# Autodesk Inventor assembly: Thigh-40x
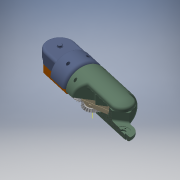
[picture p0: Inventor's stored thumbnail of the model, 180x180]
Saved by Autodesk Inventor 2018 (Build 220112000, 112)
## iProperties
Part Number: Thigh-40x
Material: Generisch
Document SubType Name: Assembly
Designer: Jochen Alt
Mass: 186.402 g
Surface Area: 1060.57 cm^2
Volume: 140.56 cm^3
Density: 1.32614 g/cm^3
Author: Jochen Alt
## Documents named in this file (12)
- D:\Projects\Manfred\design\cad\Inventor\Thigh.iam
- D:\Projects\Manfred\design\cad\Inventor\Herkulex DRS-010x\W 61707-2RS1.ipt
- D:\Projects\Manfred\design\cad\Inventor\Rillenkugellager 11x7x3 inafag smr117.ipt
- D:\Projects\Manfred\design\cad\Inventor\Thigh.ipt
- D:\Projects\Manfred\design\cad\Inventor\Herkulex DRS-040x.ipt
- D:\Projects\Manfred\design\cad\Inventor\Knee.ipt
- D:\Projects\Manfred\design\cad\Inventor\Herkulex DRS-010x\HerkuleX DRS-0101.iam
- D:\Projects\Manfred\design\cad\Inventor\Thigh Bushing.ipt
- D:\Projects\Manfred\design\cad\Inventor\ThighKneeGear.iam
- C:\Users\JochenAlt\Documents\Inventor\Content Center Files\R2018\de-DE\ISO 4762(1)\DIN EN ISO 4762 - M2 x 8.ipt
- C:\Users\JochenAlt\Documents\Inventor\Content Center Files\R2018\de-DE\ISO 4762(1)\DIN EN ISO 4762 - M2 x 6.ipt
- C:\Users\JochenAlt\Documents\Inventor\Content Center Files\R2018\de-DE\ISO 4762(1)\DIN EN ISO 4762 - M2,5 x 5.ipt
## Components (21 placed, 11 different names)
1. W 61707-2RS1:1 — Passend:44, Passend:54, Passend:73, Passend:74
2. Rillenkugellager 11x7x3 inafag smr117:2 — Passend:78, Passend:79
3. Thigh:1 — Passend:44, Passend:54, Winkel:2, Fluchtend:1, Passend:64, Winkel:3, Passend:75, Passend:77, Winkel:5, Passend:83, Einfügen:1, Einfügen:2, Einfügen:3, Einfügen:4
4. Herkulex DRS-040x:1 — Winkel:2, Fluchtend:1, Passend:64
5. Knee:1 — Passend:75, Winkel:4, Passend:82, Passend:84, Einfügen:5, Einfügen:6, Einfügen:7, Einfügen:8, Einfügen:9, Einfügen:10
6. HerkuleX DRS-0101:1 [sub-assembly] — Winkel:4, Passend:80, Passend:81
7. Thigh Bushing:1 — Passend:73, Passend:74, Passend:76, Passend:84
8. ThighKneeGear:1 [sub-assembly] — Passend:76, Passend:77, Winkel:5, Passend:78, Passend:79, Passend:80, Passend:81, Passend:82, Passend:83, Einfügen:11, Einfügen:12, Einfügen:13
9. DIN EN ISO 4762 M2,5 x 5:2 — Einfügen:1
10. DIN EN ISO 4762 M2,5 x 5:3 — Einfügen:2
11. DIN EN ISO 4762 M2,5 x 5:1 — Einfügen:3
12. DIN EN ISO 4762 M2,5 x 5:4 — Einfügen:4
13. DIN EN ISO 4762 M2 x 6:1 — Einfügen:5
14. DIN EN ISO 4762 M2 x 6:2 — Einfügen:6
15. DIN EN ISO 4762 M2 x 6:3 — Einfügen:7
16. DIN EN ISO 4762 M2 x 6:5 — Einfügen:8
17. DIN EN ISO 4762 M2 x 6:4 — Einfügen:9
18. DIN EN ISO 4762 M2 x 6:6 — Einfügen:10
19. DIN EN ISO 4762 M2 x 8:1 — Einfügen:11
20. DIN EN ISO 4762 M2 x 8:2 — Einfügen:12
21. DIN EN ISO 4762 M2 x 8:3 — Einfügen:13
## Relationships (33: Mate 15, Insert 13, Angle 4, Flush 1)
- Passend:44 [Mate]: W 61707-2RS1:1 ↔ Thigh:1
- Passend:54 [Mate]: W 61707-2RS1:1 ↔ Thigh:1
- Winkel:2 [Angle] (180 deg): Thigh:1 ↔ Herkulex DRS-040x:1
- Fluchtend:1 [Flush] (0.2 mm): Thigh:1 ↔ Herkulex DRS-040x:1
- Passend:64 [Mate]: Thigh:1 ↔ Herkulex DRS-040x:1
- Winkel:3 [Angle] (0 deg): Thigh:1
- Passend:73 [Mate]: W 61707-2RS1:1 ↔ Thigh Bushing:1
- Passend:74 [Mate] (0.1 mm): W 61707-2RS1:1 ↔ Thigh Bushing:1
- Passend:75 [Mate]: Thigh:1 ↔ Knee:1
- Winkel:4 [Angle] (180 deg): Knee:1 ↔ HerkuleX DRS-0101:1
- Passend:76 [Mate]: Thigh Bushing:1 ↔ ThighKneeGear:1
- Passend:77 [Mate] (0.1 mm): Thigh:1 ↔ ThighKneeGear:1
- Winkel:5 [Angle] (180 deg): Thigh:1 ↔ ThighKneeGear:1
- Passend:78 [Mate]: Rillenkugellager 11x7x3 inafag smr117:2 ↔ ThighKneeGear:1
- Passend:79 [Mate]: Rillenkugellager 11x7x3 inafag smr117:2 ↔ ThighKneeGear:1
- Passend:80 [Mate]: HerkuleX DRS-0101:1 ↔ ThighKneeGear:1
- Passend:81 [Mate] (0.1 mm): HerkuleX DRS-0101:1 ↔ ThighKneeGear:1
- Passend:82 [Mate]: Knee:1 ↔ ThighKneeGear:1
- Passend:83 [Mate] (0.1 mm): Thigh:1 ↔ ThighKneeGear:1
- Passend:84 [Mate]: Knee:1 ↔ Thigh Bushing:1
- Einfügen:1 [Insert]: Thigh:1 ↔ DIN EN ISO 4762 M2,5 x 5:2
- Einfügen:2 [Insert]: Thigh:1 ↔ DIN EN ISO 4762 M2,5 x 5:3
- Einfügen:3 [Insert]: Thigh:1 ↔ DIN EN ISO 4762 M2,5 x 5:1
- Einfügen:4 [Insert]: Thigh:1 ↔ DIN EN ISO 4762 M2,5 x 5:4
- Einfügen:5 [Insert]: Knee:1 ↔ DIN EN ISO 4762 M2 x 6:1
- Einfügen:6 [Insert]: Knee:1 ↔ DIN EN ISO 4762 M2 x 6:2
- Einfügen:7 [Insert]: Knee:1 ↔ DIN EN ISO 4762 M2 x 6:3
- Einfügen:8 [Insert]: Knee:1 ↔ DIN EN ISO 4762 M2 x 6:5
- Einfügen:9 [Insert]: Knee:1 ↔ DIN EN ISO 4762 M2 x 6:4
- Einfügen:10 [Insert]: Knee:1 ↔ DIN EN ISO 4762 M2 x 6:6
- Einfügen:11 [Insert]: ThighKneeGear:1 ↔ DIN EN ISO 4762 M2 x 8:1
- Einfügen:12 [Insert]: ThighKneeGear:1 ↔ DIN EN ISO 4762 M2 x 8:2
- Einfügen:13 [Insert]: ThighKneeGear:1 ↔ DIN EN ISO 4762 M2 x 8:3
